# Autodesk Inventor assembly: Stadio4
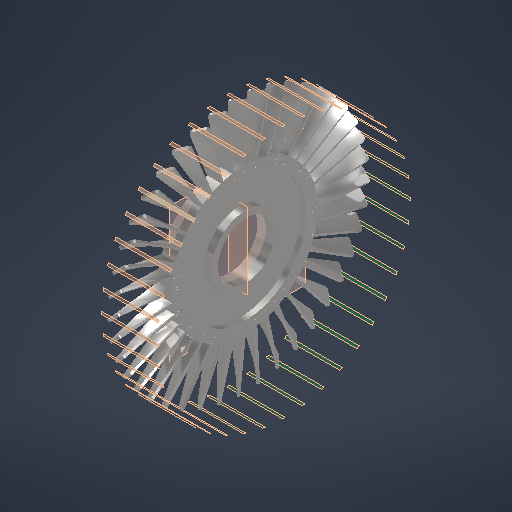
[picture p0: Inventor's stored thumbnail of the model, 512x512]
Saved by Autodesk Inventor 2026.2 (Build 302298010, 298A)
## iProperties
Created: 2026-04-23
Part Number: Stadio4
Document SubType Name: Assembly
Designer: Yan
Author: Yan
## Documents named in this file (3)
- C:\Users\Yan\Desktop\Turbina\Stadio4.iam
- C:\Users\Yan\Desktop\Turbina\DiscoPaleStadio4-DimensioniAprossimate.ipt
- C:\Users\Yan\Desktop\Turbina\PalaStadio4.ipt
## Components (41 placed, 2 different names)
1. DiscoPaleStadio4-DimensioniAprossimate:1 — Mate:1, Mate:2, Mate:3, Mate:4, Mate:5, Mate:6, Mate:7, Mate:8, Mate:9, Mate:10, Mate:11, Mate:12, Mate:13, Mate:14, Mate:15, Mate:16, Mate:17, Mate:18, Mate:19, Mate:20, Mate:21, Mate:22, Mate:23, Mate:24, Mate:25, Mate:26, Mate:27, Mate:28, Mate:29, Mate:30, Mate:31, Mate:32, Mate:33, Mate:34, Mate:35, Mate:36, Mate:37, Mate:38, Mate:40, Mate:41, Mate:42, Mate:44, Mate:45, Mate:46, Mate:47, Mate:48, Mate:49, Mate:50, Mate:51, Mate:52, Mate:53, Mate:54, Mate:55, Mate:56, Mate:57, Mate:58, Mate:59, Mate:60, Mate:61, Mate:62, Mate:63, Mate:64, Mate:65, Mate:66, Mate:67, Mate:68, Mate:69, Mate:70, Mate:71, Mate:72, Mate:73, Mate:74, Mate:75, Mate:76, Mate:77, Mate:78, Mate:79, Mate:80, Mate:81, Flush:1, Flush:2, Flush:3, Flush:4, Flush:5, Flush:6, Flush:7, Flush:8, Flush:9, Flush:10, Flush:11, Flush:12, Flush:13, Flush:14, Flush:15, Flush:16, Flush:17, Flush:18, Flush:19, Flush:20, Flush:21, Flush:22, Flush:23, Flush:24, Flush:25, Flush:26, Flush:27, Flush:28, Flush:29, Flush:30, Flush:31, Flush:32, Flush:33, Flush:34, Flush:35, Flush:36, Flush:37, Flush:38, Flush:39, Flush:40, Flush:41
2. PalaStadio4:1 — Mate:1, Mate:20, Flush:30
3. PalaStadio4:2 — Mate:2, Mate:19, Flush:29
4. PalaStadio4:3 — Mate:3, Mate:18, Flush:28
5. PalaStadio4:4 — Mate:4, Mate:17, Flush:27
6. PalaStadio4:5 — Mate:5, Mate:16, Flush:26
7. PalaStadio4:6 — Mate:6, Mate:15, Flush:25
8. PalaStadio4:7 — Mate:7, Mate:14, Flush:24
9. PalaStadio4:8 — Mate:8, Mate:13, Flush:23
10. PalaStadio4:9 — Mate:9, Mate:12, Flush:22
11. PalaStadio4:10 — Mate:10, Mate:11, Flush:21
12. PalaStadio4:11 — Mate:21, Mate:27, Flush:20
13. PalaStadio4:12 — Mate:22, Mate:28, Flush:19
14. PalaStadio4:13 — Mate:23, Mate:29, Flush:18
15. PalaStadio4:14 — Mate:24, Mate:30, Flush:17
16. PalaStadio4:15 — Mate:25, Mate:31, Flush:16
17. PalaStadio4:16 — Mate:26, Mate:34, Flush:14
18. PalaStadio4:17 — Mate:32, Mate:33, Flush:15
19. PalaStadio4:18 — Mate:35, Mate:37, Flush:13
20. PalaStadio4:19 — Mate:36, Mate:38, Flush:12
21. PalaStadio4:20 — Mate:47, Mate:48, Flush:11
22. PalaStadio4:21 — Mate:40, Mate:44, Flush:10
23. PalaStadio4:22 — Mate:41, Mate:45, Flush:9
24. PalaStadio4:23 — Mate:42, Mate:46, Flush:8
25. PalaStadio4:24 — Mate:49, Mate:81, Flush:7
26. PalaStadio4:25 — Mate:50, Mate:80, Flush:6
27. PalaStadio4:26 — Mate:51, Mate:79, Flush:5
28. PalaStadio4:27 — Mate:52, Mate:78, Flush:4
29. PalaStadio4:28 — Mate:53, Mate:77, Flush:3
30. PalaStadio4:29 — Mate:54, Flush:2
31. PalaStadio4:30 — Mate:55, Mate:76, Flush:1, Flush:41
32. PalaStadio4:31 — Mate:56, Mate:75, Flush:40
33. PalaStadio4:32 — Mate:57, Mate:74, Flush:39
34. PalaStadio4:33 — Mate:58, Mate:73, Flush:38
35. PalaStadio4:34 — Mate:59, Mate:72, Flush:37
36. PalaStadio4:35 — Mate:60, Mate:71, Flush:36
37. PalaStadio4:36 — Mate:61, Mate:70, Flush:35
38. PalaStadio4:37 — Mate:62, Mate:69, Flush:34
39. PalaStadio4:38 — Mate:63, Mate:68, Flush:33
40. PalaStadio4:39 — Mate:64, Mate:67, Flush:32
41. PalaStadio4:40 — Mate:65, Mate:66, Flush:31
## Relationships (120: Mate 79, Flush 41)
- Mate:1: DiscoPaleStadio4-DimensioniAprossimate:1 ↔ PalaStadio4:1
- Mate:2: DiscoPaleStadio4-DimensioniAprossimate:1 ↔ PalaStadio4:2
- Mate:3: DiscoPaleStadio4-DimensioniAprossimate:1 ↔ PalaStadio4:3
- Mate:4: DiscoPaleStadio4-DimensioniAprossimate:1 ↔ PalaStadio4:4
- Mate:5: DiscoPaleStadio4-DimensioniAprossimate:1 ↔ PalaStadio4:5
- Mate:6: DiscoPaleStadio4-DimensioniAprossimate:1 ↔ PalaStadio4:6
- Mate:7: DiscoPaleStadio4-DimensioniAprossimate:1 ↔ PalaStadio4:7
- Mate:8: DiscoPaleStadio4-DimensioniAprossimate:1 ↔ PalaStadio4:8
- Mate:9: DiscoPaleStadio4-DimensioniAprossimate:1 ↔ PalaStadio4:9
- Mate:10: DiscoPaleStadio4-DimensioniAprossimate:1 ↔ PalaStadio4:10
- Mate:11: DiscoPaleStadio4-DimensioniAprossimate:1 ↔ PalaStadio4:10
- Mate:12: DiscoPaleStadio4-DimensioniAprossimate:1 ↔ PalaStadio4:9
- Mate:13: DiscoPaleStadio4-DimensioniAprossimate:1 ↔ PalaStadio4:8
- Mate:14: DiscoPaleStadio4-DimensioniAprossimate:1 ↔ PalaStadio4:7
- Mate:15: DiscoPaleStadio4-DimensioniAprossimate:1 ↔ PalaStadio4:6
- Mate:16: DiscoPaleStadio4-DimensioniAprossimate:1 ↔ PalaStadio4:5
- Mate:17: DiscoPaleStadio4-DimensioniAprossimate:1 ↔ PalaStadio4:4
- Mate:18: DiscoPaleStadio4-DimensioniAprossimate:1 ↔ PalaStadio4:3
- Mate:19: DiscoPaleStadio4-DimensioniAprossimate:1 ↔ PalaStadio4:2
- Mate:20: DiscoPaleStadio4-DimensioniAprossimate:1 ↔ PalaStadio4:1
- Mate:21: DiscoPaleStadio4-DimensioniAprossimate:1 ↔ PalaStadio4:11
- Mate:22: DiscoPaleStadio4-DimensioniAprossimate:1 ↔ PalaStadio4:12
- Mate:23: DiscoPaleStadio4-DimensioniAprossimate:1 ↔ PalaStadio4:13
- Mate:24: DiscoPaleStadio4-DimensioniAprossimate:1 ↔ PalaStadio4:14
- Mate:25: DiscoPaleStadio4-DimensioniAprossimate:1 ↔ PalaStadio4:15
- Mate:26: DiscoPaleStadio4-DimensioniAprossimate:1 ↔ PalaStadio4:16
- Mate:27: DiscoPaleStadio4-DimensioniAprossimate:1 ↔ PalaStadio4:11
- Mate:28: DiscoPaleStadio4-DimensioniAprossimate:1 ↔ PalaStadio4:12
- Mate:29: DiscoPaleStadio4-DimensioniAprossimate:1 ↔ PalaStadio4:13
- Mate:30: DiscoPaleStadio4-DimensioniAprossimate:1 ↔ PalaStadio4:14
- Mate:31: DiscoPaleStadio4-DimensioniAprossimate:1 ↔ PalaStadio4:15
- Mate:32: DiscoPaleStadio4-DimensioniAprossimate:1 ↔ PalaStadio4:17
- Mate:33: DiscoPaleStadio4-DimensioniAprossimate:1 ↔ PalaStadio4:17
- Mate:34: DiscoPaleStadio4-DimensioniAprossimate:1 ↔ PalaStadio4:16
- Mate:35: DiscoPaleStadio4-DimensioniAprossimate:1 ↔ PalaStadio4:18
- Mate:36: DiscoPaleStadio4-DimensioniAprossimate:1 ↔ PalaStadio4:19
- Mate:37: DiscoPaleStadio4-DimensioniAprossimate:1 ↔ PalaStadio4:18
- Mate:38: DiscoPaleStadio4-DimensioniAprossimate:1 ↔ PalaStadio4:19
- Mate:40: DiscoPaleStadio4-DimensioniAprossimate:1 ↔ PalaStadio4:21
- Mate:41: DiscoPaleStadio4-DimensioniAprossimate:1 ↔ PalaStadio4:22
- Mate:42: DiscoPaleStadio4-DimensioniAprossimate:1 ↔ PalaStadio4:23
- Mate:44: DiscoPaleStadio4-DimensioniAprossimate:1 ↔ PalaStadio4:21
- Mate:45: DiscoPaleStadio4-DimensioniAprossimate:1 ↔ PalaStadio4:22
- Mate:46: DiscoPaleStadio4-DimensioniAprossimate:1 ↔ PalaStadio4:23
- Mate:47: DiscoPaleStadio4-DimensioniAprossimate:1 ↔ PalaStadio4:20
- Mate:48: DiscoPaleStadio4-DimensioniAprossimate:1 ↔ PalaStadio4:20
- Mate:49: DiscoPaleStadio4-DimensioniAprossimate:1 ↔ PalaStadio4:24
- Mate:50: DiscoPaleStadio4-DimensioniAprossimate:1 ↔ PalaStadio4:25
- Mate:51: DiscoPaleStadio4-DimensioniAprossimate:1 ↔ PalaStadio4:26
- Mate:52: DiscoPaleStadio4-DimensioniAprossimate:1 ↔ PalaStadio4:27
- Mate:53: DiscoPaleStadio4-DimensioniAprossimate:1 ↔ PalaStadio4:28
- Mate:54: DiscoPaleStadio4-DimensioniAprossimate:1 ↔ PalaStadio4:29
- Mate:55: DiscoPaleStadio4-DimensioniAprossimate:1 ↔ PalaStadio4:30
- Mate:56: DiscoPaleStadio4-DimensioniAprossimate:1 ↔ PalaStadio4:31
- Mate:57: DiscoPaleStadio4-DimensioniAprossimate:1 ↔ PalaStadio4:32
- Mate:58: DiscoPaleStadio4-DimensioniAprossimate:1 ↔ PalaStadio4:33
- Mate:59: DiscoPaleStadio4-DimensioniAprossimate:1 ↔ PalaStadio4:34
- Mate:60: DiscoPaleStadio4-DimensioniAprossimate:1 ↔ PalaStadio4:35
- Mate:61: DiscoPaleStadio4-DimensioniAprossimate:1 ↔ PalaStadio4:36
- Mate:62: DiscoPaleStadio4-DimensioniAprossimate:1 ↔ PalaStadio4:37
- Mate:63: DiscoPaleStadio4-DimensioniAprossimate:1 ↔ PalaStadio4:38
- Mate:64: DiscoPaleStadio4-DimensioniAprossimate:1 ↔ PalaStadio4:39
- Mate:65: DiscoPaleStadio4-DimensioniAprossimate:1 ↔ PalaStadio4:40
- Mate:66: DiscoPaleStadio4-DimensioniAprossimate:1 ↔ PalaStadio4:40
- Mate:67: DiscoPaleStadio4-DimensioniAprossimate:1 ↔ PalaStadio4:39
- Mate:68: DiscoPaleStadio4-DimensioniAprossimate:1 ↔ PalaStadio4:38
- Mate:69: DiscoPaleStadio4-DimensioniAprossimate:1 ↔ PalaStadio4:37
- Mate:70: DiscoPaleStadio4-DimensioniAprossimate:1 ↔ PalaStadio4:36
- Mate:71: DiscoPaleStadio4-DimensioniAprossimate:1 ↔ PalaStadio4:35
- Mate:72: DiscoPaleStadio4-DimensioniAprossimate:1 ↔ PalaStadio4:34
- Mate:73: DiscoPaleStadio4-DimensioniAprossimate:1 ↔ PalaStadio4:33
- Mate:74: DiscoPaleStadio4-DimensioniAprossimate:1 ↔ PalaStadio4:32
- Mate:75: DiscoPaleStadio4-DimensioniAprossimate:1 ↔ PalaStadio4:31
- Mate:76: DiscoPaleStadio4-DimensioniAprossimate:1 ↔ PalaStadio4:30
- Mate:77: DiscoPaleStadio4-DimensioniAprossimate:1 ↔ PalaStadio4:28
- Mate:78: DiscoPaleStadio4-DimensioniAprossimate:1 ↔ PalaStadio4:27
- Mate:79: DiscoPaleStadio4-DimensioniAprossimate:1 ↔ PalaStadio4:26
- Mate:80: DiscoPaleStadio4-DimensioniAprossimate:1 ↔ PalaStadio4:25
- Mate:81: DiscoPaleStadio4-DimensioniAprossimate:1 ↔ PalaStadio4:24
- Flush:1: DiscoPaleStadio4-DimensioniAprossimate:1 ↔ PalaStadio4:30
- Flush:2: DiscoPaleStadio4-DimensioniAprossimate:1 ↔ PalaStadio4:29
- Flush:3: DiscoPaleStadio4-DimensioniAprossimate:1 ↔ PalaStadio4:28
- Flush:4: DiscoPaleStadio4-DimensioniAprossimate:1 ↔ PalaStadio4:27
- Flush:5: DiscoPaleStadio4-DimensioniAprossimate:1 ↔ PalaStadio4:26
- Flush:6: DiscoPaleStadio4-DimensioniAprossimate:1 ↔ PalaStadio4:25
- Flush:7: DiscoPaleStadio4-DimensioniAprossimate:1 ↔ PalaStadio4:24
- Flush:8: DiscoPaleStadio4-DimensioniAprossimate:1 ↔ PalaStadio4:23
- Flush:9: DiscoPaleStadio4-DimensioniAprossimate:1 ↔ PalaStadio4:22
- Flush:10: DiscoPaleStadio4-DimensioniAprossimate:1 ↔ PalaStadio4:21
- Flush:11: DiscoPaleStadio4-DimensioniAprossimate:1 ↔ PalaStadio4:20
- Flush:12: DiscoPaleStadio4-DimensioniAprossimate:1 ↔ PalaStadio4:19
- Flush:13: DiscoPaleStadio4-DimensioniAprossimate:1 ↔ PalaStadio4:18
- Flush:14: DiscoPaleStadio4-DimensioniAprossimate:1 ↔ PalaStadio4:16
- Flush:15: DiscoPaleStadio4-DimensioniAprossimate:1 ↔ PalaStadio4:17
- Flush:16: DiscoPaleStadio4-DimensioniAprossimate:1 ↔ PalaStadio4:15
- Flush:17: DiscoPaleStadio4-DimensioniAprossimate:1 ↔ PalaStadio4:14
- Flush:18: DiscoPaleStadio4-DimensioniAprossimate:1 ↔ PalaStadio4:13
- Flush:19: DiscoPaleStadio4-DimensioniAprossimate:1 ↔ PalaStadio4:12
- Flush:20: DiscoPaleStadio4-DimensioniAprossimate:1 ↔ PalaStadio4:11
- Flush:21: DiscoPaleStadio4-DimensioniAprossimate:1 ↔ PalaStadio4:10
- Flush:22: DiscoPaleStadio4-DimensioniAprossimate:1 ↔ PalaStadio4:9
- Flush:23: DiscoPaleStadio4-DimensioniAprossimate:1 ↔ PalaStadio4:8
- Flush:24: DiscoPaleStadio4-DimensioniAprossimate:1 ↔ PalaStadio4:7
- Flush:25: DiscoPaleStadio4-DimensioniAprossimate:1 ↔ PalaStadio4:6
- Flush:26: DiscoPaleStadio4-DimensioniAprossimate:1 ↔ PalaStadio4:5
- Flush:27: DiscoPaleStadio4-DimensioniAprossimate:1 ↔ PalaStadio4:4
- Flush:28: DiscoPaleStadio4-DimensioniAprossimate:1 ↔ PalaStadio4:3
- Flush:29: DiscoPaleStadio4-DimensioniAprossimate:1 ↔ PalaStadio4:2
- Flush:30: DiscoPaleStadio4-DimensioniAprossimate:1 ↔ PalaStadio4:1
- Flush:31: DiscoPaleStadio4-DimensioniAprossimate:1 ↔ PalaStadio4:40
- Flush:32: DiscoPaleStadio4-DimensioniAprossimate:1 ↔ PalaStadio4:39
- Flush:33: DiscoPaleStadio4-DimensioniAprossimate:1 ↔ PalaStadio4:38
- Flush:34: DiscoPaleStadio4-DimensioniAprossimate:1 ↔ PalaStadio4:37
- Flush:35: DiscoPaleStadio4-DimensioniAprossimate:1 ↔ PalaStadio4:36
- Flush:36: DiscoPaleStadio4-DimensioniAprossimate:1 ↔ PalaStadio4:35
- Flush:37: DiscoPaleStadio4-DimensioniAprossimate:1 ↔ PalaStadio4:34
- Flush:38: DiscoPaleStadio4-DimensioniAprossimate:1 ↔ PalaStadio4:33
- Flush:39: DiscoPaleStadio4-DimensioniAprossimate:1 ↔ PalaStadio4:32
- Flush:40: DiscoPaleStadio4-DimensioniAprossimate:1 ↔ PalaStadio4:31
- Flush:41: DiscoPaleStadio4-DimensioniAprossimate:1 ↔ PalaStadio4:30
